# Autodesk Inventor assembly: 1-107
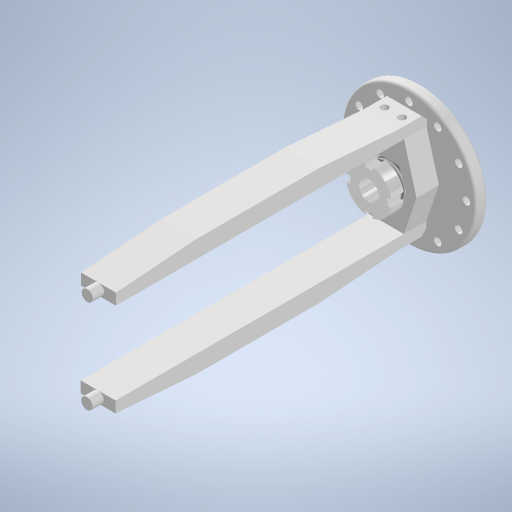
[picture p0: Inventor's stored thumbnail of the model, 512x512]
Saved by Autodesk Inventor 2024.2 (Build 282272000, 272)
## iProperties
Created: 2024-11-02
Part Number: 1-107
Document SubType Name: Assembly
Designer: Jimena Brenes
Author: Jimena Brenes
## Documents named in this file (5)
- C:\Users\Jimena Brenes\OneDrive\Escritorio\1-\1-107.iam
- C:\Users\Jimena Brenes\OneDrive\Escritorio\locomotora\1-26.ipt
- C:\Users\Jimena Brenes\OneDrive\Escritorio\PLANOS\pieza 1-29.ipt
- C:\Users\Jimena Brenes\OneDrive\Escritorio\PLANOS\pieza 1-27.ipt
- C:\Users\Jimena Brenes\OneDrive\Escritorio\PLANOS\pieza 1-28.ipt
## Components (5 placed, 4 different names)
1. 1-26:1 — Mate:1, Mate:2, Mate:3, Mate:4, Insert:1, Mate:7
2. pieza 1-29:1 — Mate:1, Mate:2
3. pieza 1-29:2 — Mate:3, Mate:4, Mate:7
4. pieza 1-27:1 — Mate:5, Mate:6, Insert:1
5. pieza 1-28:1 — Mate:5, Mate:6
## Relationships (8: Mate 7, Insert 1)
- Mate:1: 1-26:1 ↔ pieza 1-29:1
- Mate:2: 1-26:1 ↔ pieza 1-29:1
- Mate:3: 1-26:1 ↔ pieza 1-29:2
- Mate:4: 1-26:1 ↔ pieza 1-29:2
- Mate:5: pieza 1-27:1 ↔ pieza 1-28:1
- Mate:6: pieza 1-27:1 ↔ pieza 1-28:1
- Insert:1 (-5 mm): 1-26:1 ↔ pieza 1-27:1
- Mate:7: 1-26:1 ↔ pieza 1-29:2
